# Autodesk Inventor assembly: VersaPlanetary
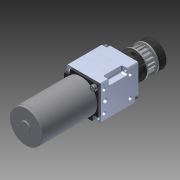
[picture p0: Inventor's stored thumbnail of the model, 180x180]
Saved by Autodesk Inventor 2014 (Build 180170000, 170)
## iProperties
Created: 2014-01-12
Part Number: VersaPlanetary
Document SubType Name: Assembly
Designer: Michael
Title: 217-1 Stage Versaplanetary STEP.STEP
Description: STEP AP214
Creation Date: 2013-12-10
Sending System: SolidWorks 2013
Preprocessor: SwSTEP 2.0
Author: Michael
## Documents named in this file (18)
- C:\Users\Andrew Toennies\Documents\GitHub\2014buildCAD\Collector\VersaPlanetary.iam
- C:\Users\Andrew Toennies\Documents\GitHub\2014buildCAD\Imported Components\217-2 Stage Versaplanetary STEP\217-2625-001 Rev1.ipt
- C:\Users\Andrew Toennies\Documents\GitHub\2014buildCAD\Imported Components\217-2 Stage Versaplanetary STEP\217-2625-002 Rev1.ipt
- C:\Users\Andrew Toennies\Documents\GitHub\2014buildCAD\Imported Components\217-2 Stage Versaplanetary STEP\217-2625-009 Rev1.ipt
- C:\Users\Andrew Toennies\Documents\GitHub\2014buildCAD\Imported Components\217-2 Stage Versaplanetary STEP\217-2816-001 Rev1.ipt
- C:\Users\Andrew Toennies\Documents\GitHub\2014buildCAD\Imported Components\217-2 Stage Versaplanetary STEP\217-2 Stage Versaplanetary STEP.iam
- C:\Users\Michael\Documents\GitHub\2014buildCAD\Imported Components\217-1 Stage Versaplanetary STEP\217-2625-012 Rev1.ipt
- C:\Users\Andrew Toennies\Documents\GitHub\2014buildCAD\Imported Components\217-2 Stage Versaplanetary STEP\SSA_SSA0832-0500ZC.ipt
- C:\Users\Andrew Toennies\Documents\GitHub\2014buildCAD\Imported Components\217-2 Stage Versaplanetary STEP\217-2742.ipt
- C:\Users\Michael\Documents\GitHub\2014buildCAD\Imported Components\217-1 Stage Versaplanetary STEP\SSA_SSA0832-1250ZC.ipt
- C:\Users\Andrew Toennies\Documents\GitHub\2014buildCAD\Imported Components\217-2 Stage Versaplanetary STEP\217-2625-018 Rev1_98541A410.ipt
- C:\Users\Andrew Toennies\Documents\GitHub\2014buildCAD\Imported Components\217-2 Stage Versaplanetary STEP\217-2625-017 Rev1_9714K61.ipt
- C:\Users\Andrew Toennies\Documents\GitHub\2014buildCAD\Imported Components\217-2 Stage Versaplanetary STEP\PINL-M020-006-S.ipt
- C:\Users\Andrew Toennies\Documents\GitHub\2014buildCAD\Collector\VersaPlanetary (1-2 in hex).ipt
- C:\Users\Andrew Toennies\Documents\GitHub\2014buildCAD\Collector\VersaPlanetary (BAG mount).ipt
- C:\Users\Andrew Toennies\Documents\GitHub\2014buildCAD\Collector\Hex Shaft Collar 1-2 in (7552K500).ipt
- C:\Users\Andrew Toennies\Documents\GitHub\2014buildCAD\Collector\Timing Pulley (HTD 5mm) - 18T 9mm Double Flange, 1-2 in Hex (VexPro).ipt
- C:\Users\Andrew Toennies\Documents\GitHub\2014buildCAD\Collector\BAG Motor.ipt
## Components (22 placed, 21 different names)
1. 217-2625-001 Rev1_1
2. 217-2625-002 Rev1_2
3. 217-2625-009 Rev1_4
4. 217-2816-001 Rev1_5
5. 217-2818 Rev1_6 [sub-assembly]
6. 217-2625-012 Rev1_7
7. SSA_SSA0832-0500ZC_8 — Insert:2
8. 217-2742_11
9. 217-2742_12 — Insert:1
10. SSA_SSA0832-1250ZC_13
11. SSA_SSA0832-1250ZC_14
12. 217-2625-018 Rev1_98541A410_15
13. 217-2625-017 Rev1_9714K61_16
14. PINL-M020-006-S_17
15. PINL-M020-006-S_18
16. SSA_SSA0832-0500ZC_20 — Insert:3
17. VersaPlanetary (1-2 in hex):1 — Insert:1, Mate:1, Mate:2, Mate:3, Mate:4, Mate:5, Mate:8, Mate:9
18. VersaPlanetary (BAG mount):1 — Insert:2, Insert:3, Insert:4, Insert:5
19. Hex Shaft Collar 1-2 in (7552K500):1 — Mate:1, Mate:2, Mate:3, Mate:6
20. Hex Shaft Collar 1-2 in (7552K500):2 — Mate:7, Mate:8, Mate:9
21. Timing Pulley (HTD 5mm) - 18T 9mm Double Flange, 1-2 in Hex (VexPro):1 — Mate:4, Mate:5, Mate:6, Mate:7
22. BAG Motor:1 — Insert:4, Insert:5
## Relationships (14: Mate 9, Insert 5)
- Insert:1: 217-2742_12 ↔ VersaPlanetary (1-2 in hex):1
- Insert:2: SSA_SSA0832-0500ZC_8 ↔ VersaPlanetary (BAG mount):1
- Insert:3: SSA_SSA0832-0500ZC_20 ↔ VersaPlanetary (BAG mount):1
- Mate:1 (4.7625 mm): VersaPlanetary (1-2 in hex):1 ↔ Hex Shaft Collar 1-2 in (7552K500):1
- Mate:2: VersaPlanetary (1-2 in hex):1 ↔ Hex Shaft Collar 1-2 in (7552K500):1
- Mate:3: VersaPlanetary (1-2 in hex):1 ↔ Hex Shaft Collar 1-2 in (7552K500):1
- Mate:4: VersaPlanetary (1-2 in hex):1 ↔ Timing Pulley (HTD 5mm) - 18T 9mm Double Flange, 1-2 in Hex (VexPro):1
- Mate:5: VersaPlanetary (1-2 in hex):1 ↔ Timing Pulley (HTD 5mm) - 18T 9mm Double Flange, 1-2 in Hex (VexPro):1
- Mate:6: Hex Shaft Collar 1-2 in (7552K500):1 ↔ Timing Pulley (HTD 5mm) - 18T 9mm Double Flange, 1-2 in Hex (VexPro):1
- Mate:7: Hex Shaft Collar 1-2 in (7552K500):2 ↔ Timing Pulley (HTD 5mm) - 18T 9mm Double Flange, 1-2 in Hex (VexPro):1
- Mate:8: VersaPlanetary (1-2 in hex):1 ↔ Hex Shaft Collar 1-2 in (7552K500):2
- Mate:9: VersaPlanetary (1-2 in hex):1 ↔ Hex Shaft Collar 1-2 in (7552K500):2
- Insert:4: VersaPlanetary (BAG mount):1 ↔ BAG Motor:1
- Insert:5: VersaPlanetary (BAG mount):1 ↔ BAG Motor:1
